# Autodesk Inventor assembly: kitchen
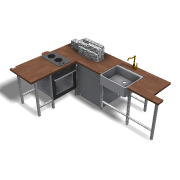
[picture p0: Inventor's stored thumbnail of the model, 180x180]
Saved by Autodesk Inventor 2018 (Build 220112000, 112)
## iProperties
Created: 2018-01-07
Part Number: kitchen
Document SubType Name: Assembly
Designer: sawaiz
Author: sawaiz
## Documents named in this file (16)
- C:\Users\sawaiz\OneDrive\projects\larkspurKitchen\frame\extrusions\kitchen.iam
- C:\Users\sawaiz\OneDrive\projects\larkspurKitchen\frame\extrusions\sinkFrame.iam
- C:\Users\sawaiz\OneDrive\projects\larkspurKitchen\appliances\sink63220001.ipt
- C:\Users\sawaiz\OneDrive\projects\larkspurKitchen\frame\extrusions\HFS5-2040-300.ipt
- C:\Users\sawaiz\OneDrive\projects\larkspurKitchen\frame\extrusions\HFS5-4040-800.ipt
- C:\Users\sawaiz\OneDrive\projects\larkspurKitchen\appliances\mieleWT946.ipt
- C:\Users\sawaiz\OneDrive\projects\larkspurKitchen\frame\extrusions\cornerFrame.iam
- C:\Users\sawaiz\OneDrive\projects\larkspurKitchen\countertop\countertopSink.ipt
- C:\Users\sawaiz\OneDrive\projects\larkspurKitchen\countertop\countertopStove.ipt
- C:\Users\sawaiz\OneDrive\projects\larkspurKitchen\frame\extrusions\HFS5-2040-500.ipt
- C:\Users\sawaiz\OneDrive\projects\larkspurKitchen\frame\extrusions\plate.iam
- C:\Users\sawaiz\OneDrive\projects\larkspurKitchen\frame\extrusions\HFS5-2040-560.ipt
- C:\Users\sawaiz\OneDrive\projects\larkspurKitchen\Cooktop.ipt
- C:\Users\sawaiz\OneDrive\projects\larkspurKitchen\appliances\samsungBF641FGB.ipt
- C:\Users\sawaiz\OneDrive\projects\larkspurKitchen\frame\extrusions\componentStack.iam
- C:\Users\sawaiz\OneDrive\projects\larkspurKitchen\appliances\hiendureBrassTap.ipt
## Components (21 placed, 15 different names)
1. sinkFrame:1 [sub-assembly] — Mate:1, Mate:2, Mate:3, Mate:4, Flush:1, Flush:2, Mate:5, Flush:3, Flush:4, Flush:7, Mate:7, Flush:8, Flush:9, Flush:10, Flush:11
2. sink63220001:1 — Mate:1, Mate:2, Mate:3
3. HFS5-2040-500:1 — Mate:4, Flush:1, Flush:2
4. HFS5-2040-500:2 — Mate:5, Flush:3, Flush:4, Flush:5, Mate:6, Flush:6
5. HFS5-4040-800:1 — Flush:5, Mate:6, Flush:6, Mate:9
6. mieleWT946:1 — Flush:7, Mate:7, Flush:8, Mate:8
7. cornerFrame:1 [sub-assembly] — Flush:9, Mate:8, Flush:10, Flush:13, Flush:14, Mate:14, Flush:17, Flush:18, Mate:15, Mate:23
8. countertopSink:1 — Mate:9, Flush:11, Mate:11, Mate:12, Flush:12, Mate:13, Mate:26, Mate:27, Mate:28
9. countertopStove:1 — Mate:11, Mate:12, Flush:12, Flush:13, Mate:22, Angle:1
10. plate:1 [sub-assembly] — Flush:14, Flush:15, Flush:16, Mate:13, Mate:16, Flush:19, Flush:20, Mate:17, Flush:21, Mate:18, Flush:22, Flush:24, Mate:19, Flush:25, Flush:26, Mate:20, Flush:28, Mate:24, Mate:25
11. plate:2 [sub-assembly] — Flush:15, Flush:16, Mate:21
12. HFS5-2040-560:1 — Flush:18, Mate:15, Mate:16, Flush:19
13. HFS5-2040-560:2 — Mate:18, Flush:22, Flush:23
14. HFS5-2040-560:3 — Mate:17, Flush:21, Flush:23, Flush:24
15. HFS5-2040-560:4 — Mate:14, Flush:17, Flush:20
16. HFS5-2040-300:1 — Flush:27, Mate:20, Flush:28, Mate:21
17. HFS5-2040-300:2 — Mate:19, Flush:25, Flush:26, Flush:27
18. Cooktop:1 — Mate:22, Angle:1
19. samsungBF641FGB:1 — Mate:23, Mate:24, Mate:25
20. componentStack:1 [sub-assembly] — Mate:26
21. hiendureBrassTap:1 — Mate:27, Mate:28
## Relationships (56: Flush 28, Mate 27, Angle 1)
- Mate:1: sinkFrame:1 ↔ sink63220001:1
- Mate:2 (2.5 mm): sinkFrame:1 ↔ sink63220001:1
- Mate:3: sinkFrame:1 ↔ sink63220001:1
- Mate:4: sinkFrame:1 ↔ HFS5-2040-500:1
- Flush:1: sinkFrame:1 ↔ HFS5-2040-500:1
- Flush:2: sinkFrame:1 ↔ HFS5-2040-500:1
- Mate:5: sinkFrame:1 ↔ HFS5-2040-500:2
- Flush:3: sinkFrame:1 ↔ HFS5-2040-500:2
- Flush:4: sinkFrame:1 ↔ HFS5-2040-500:2
- Flush:5: HFS5-2040-500:2 ↔ HFS5-4040-800:1
- Mate:6: HFS5-2040-500:2 ↔ HFS5-4040-800:1
- Flush:6: HFS5-2040-500:2 ↔ HFS5-4040-800:1
- Flush:7: sinkFrame:1 ↔ mieleWT946:1
- Mate:7 (2.5 mm): sinkFrame:1 ↔ mieleWT946:1
- Flush:8: sinkFrame:1 ↔ mieleWT946:1
- Flush:9: sinkFrame:1 ↔ cornerFrame:1
- Mate:8 (2.5 mm): mieleWT946:1 ↔ cornerFrame:1
- Flush:10: sinkFrame:1 ↔ cornerFrame:1
- Mate:9: HFS5-4040-800:1 ↔ countertopSink:1
- Flush:11 (-40 mm): sinkFrame:1 ↔ countertopSink:1
- Mate:11: countertopSink:1 ↔ countertopStove:1
- Mate:12: countertopSink:1 ↔ countertopStove:1
- Flush:12: countertopSink:1 ↔ countertopStove:1
- Flush:13 (-40 mm): cornerFrame:1 ↔ countertopStove:1
- Flush:14: cornerFrame:1 ↔ plate:1
- Flush:15: plate:1 ↔ plate:2
- Flush:16: plate:1 ↔ plate:2
- Mate:13: countertopSink:1 ↔ plate:1
- Mate:14: cornerFrame:1 ↔ HFS5-2040-560:4
- Flush:17: cornerFrame:1 ↔ HFS5-2040-560:4
- Flush:18: cornerFrame:1 ↔ HFS5-2040-560:1
- Mate:15: cornerFrame:1 ↔ HFS5-2040-560:1
- Mate:16: plate:1 ↔ HFS5-2040-560:1
- Flush:19: plate:1 ↔ HFS5-2040-560:1
- Flush:20: plate:1 ↔ HFS5-2040-560:4
- Mate:17: plate:1 ↔ HFS5-2040-560:3
- Flush:21: plate:1 ↔ HFS5-2040-560:3
- Mate:18: plate:1 ↔ HFS5-2040-560:2
- Flush:22: plate:1 ↔ HFS5-2040-560:2
- Flush:23: HFS5-2040-560:2 ↔ HFS5-2040-560:3
- Flush:24: plate:1 ↔ HFS5-2040-560:3
- Mate:19: plate:1 ↔ HFS5-2040-300:2
- Flush:25: plate:1 ↔ HFS5-2040-300:2
- Flush:26: plate:1 ↔ HFS5-2040-300:2
- Flush:27: HFS5-2040-300:1 ↔ HFS5-2040-300:2
- Mate:20: plate:1 ↔ HFS5-2040-300:1
- Flush:28: plate:1 ↔ HFS5-2040-300:1
- Mate:21: plate:2 ↔ HFS5-2040-300:1
- Mate:22: countertopStove:1 ↔ Cooktop:1
- Angle:1 (180 deg): countertopStove:1 ↔ Cooktop:1
- Mate:23 (2.5 mm): cornerFrame:1 ↔ samsungBF641FGB:1
- Mate:24: plate:1 ↔ samsungBF641FGB:1
- Mate:25: plate:1 ↔ samsungBF641FGB:1
- Mate:26: countertopSink:1 ↔ componentStack:1
- Mate:27: countertopSink:1 ↔ hiendureBrassTap:1
- Mate:28: countertopSink:1 ↔ hiendureBrassTap:1
